# Autodesk Inventor assembly: Assembly1
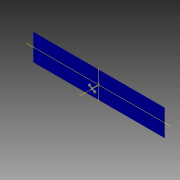
[picture p0: Inventor's stored thumbnail of the model, 180x180]
Saved by Autodesk Inventor 2014 (Build 180170000, 170)
## iProperties
Created: 2015-04-22
Part Number: Assembly1
Document SubType Name: Assembly
Designer: Vladyslav
Author: Vladyslav
## Documents named in this file (3)
- D:\Documents\Inventor\Lab9\Assembly1.iam
- D:\Documents\Inventor\Lab9\wall.ipt
- D:\Documents\Inventor\Lab9\weight.ipt
## Components (2 placed, 2 different names)
1. wall:1 — Mate:1, Mate:2, Mate:3, Mate:4
2. weight:1 — Mate:5, Angle:1
## Relationships (6: Mate 5, Angle 1)
- Mate:1: wall:1
- Mate:2: wall:1
- Mate:3: wall:1
- Mate:4: wall:1
- Mate:5: weight:1
- Angle:1 (-90 deg): weight:1
## Named parameters: angle = -90 deg
